# Autodesk Inventor assembly: Matchboxscope_v1
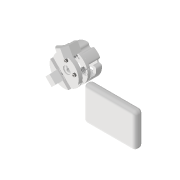
[picture p0: Inventor's stored thumbnail of the model, 180x180]
Saved by Autodesk Inventor 2022 (Build 260153000, 153)
## iProperties
Created: 2022-04-02
Part Number: Matchboxscope_v1
Document SubType Name: Assembly
Designer: Prakash Lab
Author: Prakash Lab
## Documents named in this file (11)
- C:\Users\diederichbenedict\Dropbox\Dokumente\Promotion\PROJECTS\Matchboxscope\INVENTOR\Matchboxscope_v1.iam
- C:\Users\diederichbenedict\Dropbox\Dokumente\Promotion\PROJECTS\Matchboxscope\INVENTOR\Matchboxscope_middle2_v1.ipt
- C:\Users\diederichbenedict\Dropbox\Dokumente\Promotion\PROJECTS\Matchboxscope\INVENTOR\Matchboxscope_Lightperiscope_V0.ipt
- C:\Users\diederichbenedict\Dropbox\Dokumente\Promotion\PROJECTS\Matchboxscope\INVENTOR\Matchboxscope_Lightperiscope_long_V0.ipt
- C:\Users\diederichbenedict\Dropbox\Dokumente\Promotion\PROJECTS\Matchboxscope\INVENTOR\Matchboxscope_bottom_v0.ipt
- C:\Users\diederichbenedict\Dropbox\Dokumente\Promotion\PROJECTS\Matchboxscope\INVENTOR\00_ESP3-CAM.iam
- C:\Users\diederichbenedict\Dropbox\Dokumente\Promotion\PROJECTS\Matchboxscope\INVENTOR\Matchboxscope_sample_v1.ipt
- C:\Users\diederichbenedict\Dropbox\Dokumente\Promotion\PROJECTS\Matchboxscope\INVENTOR\Matchboxscope_lenstube_v0.ipt
- C:\Users\diederichbenedict\Dropbox\Dokumente\Promotion\PROJECTS\Matchboxscope\INVENTOR\00_Powerbank.ipt
- C:\Users\diederichbenedict\Dropbox\Dokumente\Promotion\PROJECTS\Matchboxscope\INVENTOR\00_spring.ipt
- C:\Users\diederichbenedict\Documents\Inventor\Content Center Files\R2022\de-DE\DIN 912\DIN 912 - M3 x 0.5 x 25 x 18.ipt
## Components (14 placed, 10 different names)
1. Matchboxscope_middle2_v1:1 — Insert:1, Angle:1, Mate:5, Flush:2, Flush:3, Einfügen:3, Passend:7
2. Matchboxscope_Lightperiscope_V0:1
3. Matchboxscope_Lightperiscope_long_V0:1 — Insert:2, Angle:2, Einfügen:10
4. Matchboxscope_bottom_v0:1 — Mate:1, Mate:2, Mate:3, Mate:4, Flush:1, Mate:5
5. 00_ESP3-CAM:1 [sub-assembly] — Mate:4, Flush:1, Insert:1
6. Matchboxscope_sample_v1:1 — Flush:2, Flush:3, Insert:2, Angle:2, Mate:6, Einfügen:4, Einfügen:5, Einfügen:6, Einfügen:7, Einfügen:8, Einfügen:9, Einfügen:10
7. Matchboxscope_lenstube_v0:1 — Mate:6, Einfügen:3
8. 00_Powerbank:1
9. 00_spring:1 — Einfügen:9
10. DIN 912 - ersetzt durch DIN EN ISO 4762 M3 x 25:1 — Einfügen:6, Passend:7
11. DIN 912 - ersetzt durch DIN EN ISO 4762 M3 x 25:2 — Einfügen:5
12. DIN 912 - ersetzt durch DIN EN ISO 4762 M3 x 25:3 — Einfügen:4
13. 00_spring:3 — Einfügen:7
14. 00_spring:4 — Einfügen:8
## Relationships (22: Insert 10, Mate 7, Flush 3, Angle 2)
- Mate:1: Matchboxscope_bottom_v0:1
- Mate:2: Matchboxscope_bottom_v0:1
- Mate:3: Matchboxscope_bottom_v0:1
- Mate:4: Matchboxscope_bottom_v0:1 ↔ 00_ESP3-CAM:1
- Flush:1: Matchboxscope_bottom_v0:1 ↔ 00_ESP3-CAM:1
- Insert:1: Matchboxscope_middle2_v1:1 ↔ 00_ESP3-CAM:1
- Angle:1 (0 deg): Matchboxscope_middle2_v1:1
- Mate:5: Matchboxscope_middle2_v1:1 ↔ Matchboxscope_bottom_v0:1
- Flush:2: Matchboxscope_middle2_v1:1 ↔ Matchboxscope_sample_v1:1
- Flush:3: Matchboxscope_middle2_v1:1 ↔ Matchboxscope_sample_v1:1
- Insert:2 (-3 mm): Matchboxscope_Lightperiscope_long_V0:1 ↔ Matchboxscope_sample_v1:1
- Angle:2 (90 deg): Matchboxscope_Lightperiscope_long_V0:1 ↔ Matchboxscope_sample_v1:1
- Mate:6: Matchboxscope_sample_v1:1 ↔ Matchboxscope_lenstube_v0:1
- Einfügen:3 [Insert]: Matchboxscope_middle2_v1:1 ↔ Matchboxscope_lenstube_v0:1
- Einfügen:4 [Insert]: Matchboxscope_sample_v1:1 ↔ DIN 912 - ersetzt durch DIN EN ISO 4762 M3 x 25:3
- Einfügen:5 [Insert]: Matchboxscope_sample_v1:1 ↔ DIN 912 - ersetzt durch DIN EN ISO 4762 M3 x 25:2
- Einfügen:6 [Insert]: Matchboxscope_sample_v1:1 ↔ DIN 912 - ersetzt durch DIN EN ISO 4762 M3 x 25:1
- Einfügen:7 [Insert]: Matchboxscope_sample_v1:1 ↔ 00_spring:3
- Einfügen:8 [Insert]: Matchboxscope_sample_v1:1 ↔ 00_spring:4
- Einfügen:9 [Insert]: Matchboxscope_sample_v1:1 ↔ 00_spring:1
- Passend:7 [Mate]: Matchboxscope_middle2_v1:1 ↔ DIN 912 - ersetzt durch DIN EN ISO 4762 M3 x 25:1
- Einfügen:10 [Insert]: Matchboxscope_Lightperiscope_long_V0:1 ↔ Matchboxscope_sample_v1:1
